# Autodesk Inventor assembly: Robot
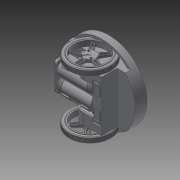
[picture p0: Inventor's stored thumbnail of the model, 180x180]
Saved by Autodesk Inventor 2014 (Build 180170000, 170)
## iProperties
Created: 2013-06-25
Part Number: Robot
Document SubType Name: Assembly
Designer: Felix
Author: Felix
## Documents named in this file (8)
- C:\Users\hanse\Desktop\Beep\Hardware\3D-CAD\Robot.iam
- C:\Users\hanse\Desktop\Beep\Hardware\3D-CAD\Pololu_gear_motor_1_180\gear_motor.iam
- C:\Users\hanse\Desktop\Beep\Hardware\3D-CAD\Pololu_Wheel_6mm\Wheel.iam
- C:\Users\hanse\Desktop\Beep\Hardware\3D-CAD\battery_holder\holder_with_batteries_18500.iam
- C:\Users\hanse\Desktop\Beep\Hardware\3D-CAD\battery_holder\holder_with_batteries_18650.iam
- C:\Users\Felix\Documents\Inventor\Content Center Files\R2014\de-DE\ISO 7046-1(1)\ISO 7046-1 - M2 x 8 - 4.8 - HDIN EN ISO.ipt
- C:\Users\hanse\Desktop\Beep\Hardware\3D-CAD\case\base.ipt
- C:\Users\hanse\Desktop\Beep\Hardware\3D-CAD\RaspberryPi\RaspberryPi.iam
## Components (10 placed, 7 different names)
1. gear_motor:1 [sub-assembly] — Passend:1, Passend:5, Passend:6, Passend:7, Fluchtend:3, Passend:13, Passend:14, Passend:16, Passend:18, Passend:19, Passend:24
2. gear_motor:2 [sub-assembly] — Passend:1, Passend:2, Passend:3, Passend:4, Fluchtend:3, Fluchtend:4, Fluchtend:5, Passend:12, Passend:15
3. Wheel:1 [sub-assembly] — Passend:5, Passend:6, Passend:7, Passend:24
4. Wheel:2 [sub-assembly] — Passend:2, Passend:3, Passend:4
5. holder_with_batteries_18500:1 [sub-assembly] — Fluchtend:4, Passend:13, Passend:14, Passend:15, Fluchtend:6
6. holder_with_batteries_18650:1 [sub-assembly] — Fluchtend:5, Passend:12, Passend:16, Passend:20, Passend:21, Passend:22, Passend:23
7. DIN EN ISO 7046-1 H M2 x 8 - 4.8 - H:1 — Passend:20, Passend:23
8. DIN EN ISO 7046-1 H M2 x 8 - 4.8 - H:2 — Passend:21, Passend:22
9. base:1 — Fluchtend:6, Passend:25
10. RaspberryPi:1 [sub-assembly] — Passend:25
## Relationships (24: Mate 20, Flush 4)
- Passend:1 [Mate]: gear_motor:1 ↔ gear_motor:2
- Passend:2 [Mate]: gear_motor:2 ↔ Wheel:2
- Passend:3 [Mate]: gear_motor:2 ↔ Wheel:2
- Passend:4 [Mate]: gear_motor:2 ↔ Wheel:2
- Passend:5 [Mate]: gear_motor:1 ↔ Wheel:1
- Passend:6 [Mate]: gear_motor:1 ↔ Wheel:1
- Passend:7 [Mate]: gear_motor:1 ↔ Wheel:1
- Fluchtend:3 [Flush]: gear_motor:1 ↔ gear_motor:2
- Fluchtend:4 [Flush]: gear_motor:2 ↔ holder_with_batteries_18500:1
- Fluchtend:5 [Flush]: gear_motor:2 ↔ holder_with_batteries_18650:1
- Passend:12 [Mate]: gear_motor:2 ↔ holder_with_batteries_18650:1
- Passend:13 [Mate]: gear_motor:1 ↔ holder_with_batteries_18500:1
- Passend:14 [Mate]: gear_motor:1 ↔ holder_with_batteries_18500:1
- Passend:15 [Mate]: gear_motor:2 ↔ holder_with_batteries_18500:1
- Passend:16 [Mate]: gear_motor:1 ↔ holder_with_batteries_18650:1
- Passend:18 [Mate]: gear_motor:1
- Passend:19 [Mate]: gear_motor:1
- Passend:20 [Mate]: holder_with_batteries_18650:1 ↔ DIN EN ISO 7046-1 H M2 x 8 - 4.8 - H:1
- Passend:21 [Mate]: holder_with_batteries_18650:1 ↔ DIN EN ISO 7046-1 H M2 x 8 - 4.8 - H:2
- Passend:22 [Mate]: holder_with_batteries_18650:1 ↔ DIN EN ISO 7046-1 H M2 x 8 - 4.8 - H:2
- Passend:23 [Mate]: holder_with_batteries_18650:1 ↔ DIN EN ISO 7046-1 H M2 x 8 - 4.8 - H:1
- Passend:24 [Mate]: gear_motor:1 ↔ Wheel:1
- Fluchtend:6 [Flush]: holder_with_batteries_18500:1 ↔ base:1
- Passend:25 [Mate]: base:1 ↔ RaspberryPi:1
